# Autodesk Inventor assembly: SeatModuleSubassembly
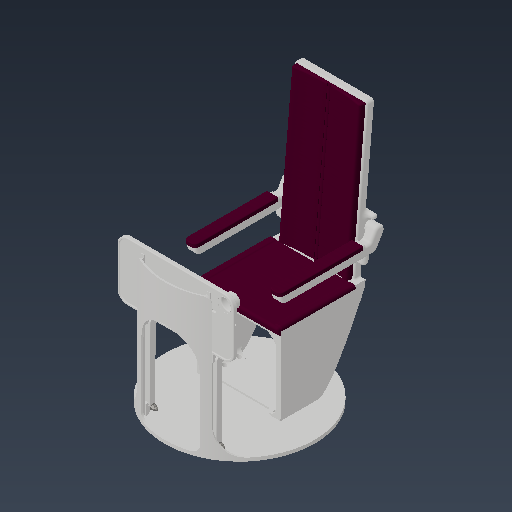
[picture p0: Inventor's stored thumbnail of the model, 512x512]
Saved by Autodesk Inventor 2021 (Build 250183000, 183)
## iProperties
Created: 2021-01-30
Part Number: SeatModuleSubassembly
Document SubType Name: Assembly
Designer: argon
Author: argon
## Documents named in this file (4)
- C:\Users\argon\OneDrive\Documents\GrabCAD\EngOne Maroons\Seat Module Subassembly\SeatModuleSubassembly.iam
- C:\Users\argon\OneDrive\Documents\GrabCAD\EngOne Maroons\Seat Module Subassembly\Baseplate.ipt
- C:\Users\argon\OneDrive\Documents\GrabCAD\EngOne Maroons\Seat Subassembly\SeatSubassembly.iam
- C:\Users\argon\OneDrive\Documents\GrabCAD\EngOne Maroons\Table Subassemly\Table Subassembly.iam
## Components (3 placed, 3 different names)
1. Baseplate:1 — Mate:1, Mate:2, Mate:3, Mate:4, Mate:5, Mate:6, Mate:7
2. SeatSubassembly:1 [sub-assembly] — Mate:1, Mate:2, Mate:3
3. Table Subassembly:1 [sub-assembly] — Mate:4, Mate:5, Mate:6, Mate:7
## Relationships (7: Mate 7)
- Mate:1: Baseplate:1 ↔ SeatSubassembly:1
- Mate:2: Baseplate:1 ↔ SeatSubassembly:1
- Mate:3: Baseplate:1 ↔ SeatSubassembly:1
- Mate:4: Baseplate:1 ↔ Table Subassembly:1
- Mate:5: Baseplate:1 ↔ Table Subassembly:1
- Mate:6: Baseplate:1 ↔ Table Subassembly:1
- Mate:7: Baseplate:1 ↔ Table Subassembly:1
